# Autodesk Inventor assembly: Assembly1
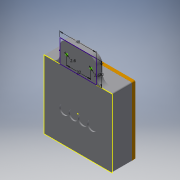
[picture p0: Inventor's stored thumbnail of the model, 180x180]
Saved by Autodesk Inventor 2019 (Build 230136000, 136)
## iProperties
Created: 2021-10-12
Part Number: Assembly1
Document SubType Name: Assembly
Designer: Pulag
Author: Pulag
## Documents named in this file (4)
- C:\Users\Pulag\Desktop\project\not_drawing_sys_2.0\cad\Assembly1.iam
- C:\Users\Pulag\Desktop\project\not_drawing_sys_2.0\cad\base.ipt
- C:\Users\Pulag\Desktop\project\not_drawing_sys_2.0\cad\covor.ipt
- C:\Users\Pulag\Desktop\project\not_drawing_sys_2.0\cad\but.ipt
## Components (3 placed, 3 different names)
1. base:1 — Flush:1
2. covor:1 — Flush:1, Mate:1, Mate:2
3. but:1 — Mate:1, Mate:2
## Relationships (3: Mate 2, Flush 1)
- Flush:1 (3 mm): base:1 ↔ covor:1
- Mate:1: covor:1 ↔ but:1
- Mate:2 (-5.78 mm): covor:1 ↔ but:1
